# Autodesk Inventor assembly: Tenor Cart
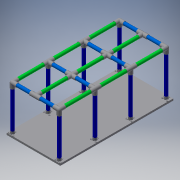
[picture p0: Inventor's stored thumbnail of the model, 180x180]
Saved by Autodesk Inventor 2018.2 (Build 222227000, 227)
## iProperties
Created: 2018-03-15
Part Number: Tenor Cart
Document SubType Name: Assembly
Designer: owner
Author: owner
## Documents named in this file (10)
- Z:\The Pickle\Final Carts\Sax Cart\Tenor Cart.iam
- Z:\The Pickle\Final Carts\Sax Cart\Tenor Base.ipt
- Z:\The Pickle\Final Carts\Sax Cart\Pipe 5.ipt
- Z:\The Pickle\Final Carts\Sax Cart\Pipe 1.ipt
- Z:\The Pickle\Final Carts\Sax Cart\Pipe 2.ipt
- Z:\The Pickle\Inventor Pipe Parts\Formufit Fittings\Wood Mount 1 Inch.ipt
- Z:\The Pickle\Inventor Pipe Parts\Formufit Fittings\3-way 90 1 Inch.ipt
- Z:\The Pickle\Inventor Pipe Parts\Formufit Fittings\4-way Tee 1 Inch.ipt
- Z:\The Pickle\Inventor Pipe Parts\Formufit Fittings\Tee 1 Inch.ipt
- Z:\The Pickle\Inventor Pipe Parts\Formufit Fittings\Cross 1 Inch.ipt
## Components (46 placed, 9 different names)
1. Tenor Base:1 — Mate:1, Tangent:1, Tangent:2, Tangent:3
2. Pipe 5:1 — Insert:10, Insert:11
3. Pipe 5:2 — Insert:13, Insert:14
4. Pipe 5:3 — Insert:22, Insert:23
5. Pipe 5:4 — Insert:24, Insert:29
6. Pipe 5:5 — Insert:35, Insert:36
7. Pipe 5:6 — Insert:38
8. Pipe 5:7 — Insert:41, Insert:42
9. Pipe 5:8 — Insert:43, Insert:44
10. Pipe 1:1 — Insert:1, Insert:9
11. Pipe 1:2 — Insert:2, Insert:15
12. Pipe 1:3 — Insert:3, Insert:18
13. Pipe 1:4 — Insert:8, Insert:19
14. Pipe 1:5 — Insert:5, Insert:26
15. Pipe 1:6 — Insert:6, Insert:27
16. Pipe 1:7 — Insert:7, Insert:28
17. Pipe 2:1 — Insert:30
18. Pipe 2:2 — Insert:12
19. Pipe 2:3 — Insert:16, Insert:17
20. Pipe 2:4 — Insert:20, Insert:21
21. Pipe 2:5 — Insert:37
22. Pipe 2:6 — Insert:31, Insert:32
23. Pipe 2:7 — Insert:33, Insert:34
24. Pipe 2:8 — Insert:40
25. Pipe 2:9 — Insert:39
26. Pipe 1:8 — Insert:4, Insert:25
27. Wood Mount 1 Inch:1 — Flush:7, Mate:1, Tangent:1, Tangent:2, Tangent:3, Insert:1
28. Wood Mount 1 Inch:2 — Flush:6, Flush:7, Insert:4
29. Wood Mount 1 Inch:3 — Flush:5, Flush:6, Insert:5
30. Wood Mount 1 Inch:4 — Flush:4, Flush:5, Insert:6
31. Wood Mount 1 Inch:5 — Flush:3, Flush:4, Insert:7
32. Wood Mount 1 Inch:6 — Flush:2, Flush:3, Insert:8
33. Wood Mount 1 Inch:7 — Flush:1, Flush:2, Insert:3
34. Wood Mount 1 Inch:8 — Flush:1, Insert:2
35. 3-way 90 1 Inch:1 — Insert:14, Insert:15, Insert:16
36. 3-way 90 1 Inch:2 — Insert:28, Insert:44
37. 3-way 90 1 Inch:3 — Insert:27, Insert:34, Insert:41
38. 3-way 90 1 Inch:4 — Insert:9, Insert:10, Insert:30
39. 4-way Tee 1 Inch:1 — Insert:25, Insert:29, Insert:31
40. 4-way Tee 1 Inch:2 — Insert:26, Insert:32, Insert:33, Insert:35
41. 4-way Tee 1 Inch:3 — Insert:17, Insert:18, Insert:20, Insert:22
42. 4-way Tee 1 Inch:4 — Insert:19, Insert:21, Insert:39
43. Tee 1 Inch:1 — Insert:11, Insert:12, Insert:13
44. Tee 1 Inch:2 — Insert:42, Insert:43
45. Cross 1 Inch:1 — Insert:36, Insert:38, Insert:40
46. Cross 1 Inch:2 — Insert:23, Insert:24, Insert:37
## Relationships (55: Insert 44, Flush 7, Tangent 3, Mate 1)
- Flush:1: Wood Mount 1 Inch:7 ↔ Wood Mount 1 Inch:8
- Flush:2: Wood Mount 1 Inch:6 ↔ Wood Mount 1 Inch:7
- Flush:3: Wood Mount 1 Inch:5 ↔ Wood Mount 1 Inch:6
- Flush:4: Wood Mount 1 Inch:4 ↔ Wood Mount 1 Inch:5
- Flush:5: Wood Mount 1 Inch:3 ↔ Wood Mount 1 Inch:4
- Flush:6: Wood Mount 1 Inch:2 ↔ Wood Mount 1 Inch:3
- Flush:7: Wood Mount 1 Inch:1 ↔ Wood Mount 1 Inch:2
- Mate:1: Tenor Base:1 ↔ Wood Mount 1 Inch:1
- Tangent:1: Tenor Base:1 ↔ Wood Mount 1 Inch:1
- Tangent:2: Tenor Base:1 ↔ Wood Mount 1 Inch:1
- Tangent:3: Tenor Base:1 ↔ Wood Mount 1 Inch:1
- Insert:1: Pipe 1:1 ↔ Wood Mount 1 Inch:1
- Insert:2: Pipe 1:2 ↔ Wood Mount 1 Inch:8
- Insert:3: Pipe 1:3 ↔ Wood Mount 1 Inch:7
- Insert:4: Pipe 1:8 ↔ Wood Mount 1 Inch:2
- Insert:5: Pipe 1:5 ↔ Wood Mount 1 Inch:3
- Insert:6: Pipe 1:6 ↔ Wood Mount 1 Inch:4
- Insert:7: Pipe 1:7 ↔ Wood Mount 1 Inch:5
- Insert:8: Pipe 1:4 ↔ Wood Mount 1 Inch:6
- Insert:9: Pipe 1:1 ↔ 3-way 90 1 Inch:4
- Insert:10: Pipe 5:1 ↔ 3-way 90 1 Inch:4
- Insert:11: Pipe 5:1 ↔ Tee 1 Inch:1
- Insert:12: Pipe 2:2 ↔ Tee 1 Inch:1
- Insert:13: Pipe 5:2 ↔ Tee 1 Inch:1
- Insert:14: Pipe 5:2 ↔ 3-way 90 1 Inch:1
- Insert:15: Pipe 1:2 ↔ 3-way 90 1 Inch:1
- Insert:16: Pipe 2:3 ↔ 3-way 90 1 Inch:1
- Insert:17: Pipe 2:3 ↔ 4-way Tee 1 Inch:3
- Insert:18: Pipe 1:3 ↔ 4-way Tee 1 Inch:3
- Insert:19: Pipe 1:4 ↔ 4-way Tee 1 Inch:4
- Insert:20: Pipe 2:4 ↔ 4-way Tee 1 Inch:3
- Insert:21: Pipe 2:4 ↔ 4-way Tee 1 Inch:4
- Insert:22: Pipe 5:3 ↔ 4-way Tee 1 Inch:3
- Insert:23: Pipe 5:3 ↔ Cross 1 Inch:2
- Insert:24: Pipe 5:4 ↔ Cross 1 Inch:2
- Insert:25: Pipe 1:8 ↔ 4-way Tee 1 Inch:1
- Insert:26: Pipe 1:5 ↔ 4-way Tee 1 Inch:2
- Insert:27: Pipe 1:6 ↔ 3-way 90 1 Inch:3
- Insert:28: Pipe 1:7 ↔ 3-way 90 1 Inch:2
- Insert:29: Pipe 5:4 ↔ 4-way Tee 1 Inch:1
- Insert:30: Pipe 2:1 ↔ 3-way 90 1 Inch:4
- Insert:31: Pipe 2:6 ↔ 4-way Tee 1 Inch:1
- Insert:32: Pipe 2:6 ↔ 4-way Tee 1 Inch:2
- Insert:33: Pipe 2:7 ↔ 4-way Tee 1 Inch:2
- Insert:34: Pipe 2:7 ↔ 3-way 90 1 Inch:3
- Insert:35: Pipe 5:5 ↔ 4-way Tee 1 Inch:2
- Insert:36: Pipe 5:5 ↔ Cross 1 Inch:1
- Insert:37: Pipe 2:5 ↔ Cross 1 Inch:2
- Insert:38: Pipe 5:6 ↔ Cross 1 Inch:1
- Insert:39: Pipe 2:9 ↔ 4-way Tee 1 Inch:4
- Insert:40: Pipe 2:8 ↔ Cross 1 Inch:1
- Insert:41: Pipe 5:7 ↔ 3-way 90 1 Inch:3
- Insert:42: Pipe 5:7 ↔ Tee 1 Inch:2
- Insert:43: Pipe 5:8 ↔ Tee 1 Inch:2
- Insert:44: Pipe 5:8 ↔ 3-way 90 1 Inch:2
